# Autodesk Inventor assembly: 03_XY_Assy
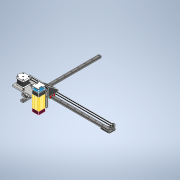
[picture p0: Inventor's stored thumbnail of the model, 180x180]
Saved by Autodesk Inventor 2022.2 (Build 262287010, 287A)
## iProperties
Created: 2022-05-03
Part Number: 03_XY_Assy
Document SubType Name: Assembly
Designer: MXBD
Author: MXBD
## Documents named in this file (5)
- D:\Laser_Engraver\CAD\Assembly\03_XY_Assy.iam
- D:\Laser_Engraver\CAD\Assembly\00_Linear_rail_Y.iam
- D:\Laser_Engraver\CAD\Assembly\00_Linear_rail_X.iam
- C:\Users\49152\Documents\Inventor\Content Center Files\R2022\de-DE\ISO 4035(1)\ISO 4035 - M3DIN EN.ipt
- C:\Users\49152\Documents\Inventor\Content Center Files\R2022\de-DE\ISO 4762(2)\ISO 4762 - M3 x 16ISO.ipt
## Components (6 placed, 4 different names)
1. 00_Linear_rail_Y:1 [sub-assembly] — Passend:1, Passend:2, Passend:3, Passend:4, Passend:5, Passend:6, Passend:7
2. 00_Linear_rail_X:1 [sub-assembly] — Passend:1, Passend:2, Passend:3, Passend:8, Passend:9, Passend:10, Passend:11
3. DIN EN 24035 M3:1 — Passend:4, Passend:6
4. DIN EN 24035 M3:2 — Passend:5, Passend:7
5. ISO 4762 M3 x 16:1 — Passend:8, Passend:11
6. ISO 4762 M3 x 16:2 — Passend:9, Passend:10
## Relationships (11: Mate 11)
- Passend:1 [Mate]: 00_Linear_rail_Y:1 ↔ 00_Linear_rail_X:1
- Passend:2 [Mate]: 00_Linear_rail_Y:1 ↔ 00_Linear_rail_X:1
- Passend:3 [Mate]: 00_Linear_rail_Y:1 ↔ 00_Linear_rail_X:1
- Passend:4 [Mate]: 00_Linear_rail_Y:1 ↔ DIN EN 24035 M3:1
- Passend:5 [Mate]: 00_Linear_rail_Y:1 ↔ DIN EN 24035 M3:2
- Passend:6 [Mate]: 00_Linear_rail_Y:1 ↔ DIN EN 24035 M3:1
- Passend:7 [Mate]: 00_Linear_rail_Y:1 ↔ DIN EN 24035 M3:2
- Passend:8 [Mate]: 00_Linear_rail_X:1 ↔ ISO 4762 M3 x 16:1
- Passend:9 [Mate]: 00_Linear_rail_X:1 ↔ ISO 4762 M3 x 16:2
- Passend:10 [Mate]: 00_Linear_rail_X:1 ↔ ISO 4762 M3 x 16:2
- Passend:11 [Mate]: 00_Linear_rail_X:1 ↔ ISO 4762 M3 x 16:1
